# Autodesk Inventor assembly: pld-octogon
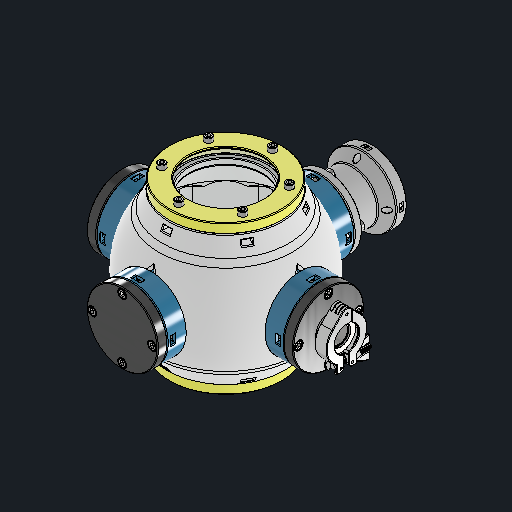
[picture p0: Inventor's stored thumbnail of the model, 512x512]
Saved by Autodesk Inventor 2026 (Build 300175050, 175E)
## iProperties
Created: 2025-12-11
Part Number: pld-octogon
Document SubType Name: Assembly
Designer: kuzmin
Author: kuzmin
## Documents named in this file (11)
- C:\Users\queezz\Dropbox\Drawings\PIHTI\PLD\pld-octogon.iam
- C:\Users\queezz\Dropbox\Drawings\PIHTI\PLD\pld-octogon.ipt
- C:\Users\queezz\Dropbox\Drawings\PIHTI\PLD\pld-octogon-nipple.ipt
- C:\Users\queezz\Dropbox\Drawings\PIHTI\PLD\oring-60-68.ipt
- C:\Users\queezz\Dropbox\Drawings\PIHTI\PLD\pld_nipple-70mm.iam
- C:\Users\queezz\Dropbox\Drawings\PIHTI\ContentCenter\Fastners\M6-nut-WA5.ipt
- C:\Users\queezz\Dropbox\Drawings\PIHTI\ContentCenter\Fastners\M6x25-SHCS.ipt
- C:\Users\queezz\Dropbox\Drawings\PIHTI\PLD\oring-102-110.ipt
- C:\Users\queezz\Dropbox\Drawings\PIHTI\PLD\akf-100-window.iam
- C:\Users\queezz\Dropbox\Drawings\PIHTI\PLD\akf-60-blank.ipt
- C:\Users\queezz\Dropbox\Drawings\PIHTI\PLD\akf-60-nw25.iam
## Components (47 placed, 10 different names)
1. pld-octogon:1 — Rigid:1, Flush:1, Flush:2, Mate:1, Rigid:3, Rigid:4, Rigid:5, Rigid:18, Rigid:19, Rigid:26, Rotational:1, Rigid:33, Rigid:34, Rigid:35, Rigid:36, Rigid:37, Rigid:38
2. pld-octogon-nipple:1 — Rigid:1, Rigid:6, Mate:2, Mate:3
3. pld-octogon-nipple:2 — Rigid:3
4. pld-octogon-nipple:3 — Rigid:4
5. pld-octogon-nipple:4 — Rigid:5
6. oring-60-68:1 — Rigid:6, Tangent:1
7. oring-60-68:2
8. oring-60-68:3
9. oring-60-68:4
10. pld_nipple-70mm:1 [sub-assembly] — Mate:2, Mate:3, Tangent:1, Rigid:14, Rigid:15, Rigid:16, Rigid:17
11. oring-102-110:1 — Rigid:18
12. akf-100-window:2 [sub-assembly] — Rigid:19, Rigid:20, Rigid:21, Rigid:22, Rigid:23, Rigid:24, Rigid:25
13. akf-100-window:3 [sub-assembly] — Rotational:1, Rigid:27, Rigid:28, Rigid:29, Rigid:30, Rigid:31, Rigid:32
14. oring-102-110:2 — Rigid:26
15. akf-60-blank:2 — Rigid:44, Rigid:45, Rigid:46, Rigid:47
16. akf-60-blank:3
17. akf-60-nw25:2 [sub-assembly]
18. IS 2269 M6 x 25:17 — Rigid:47
19. IS 2269 M6 x 25:18 — Rigid:44
20. IS 2269 M6 x 25:19 — Rigid:46
21. IS 2269 M6 x 25:20 — Rigid:45
22. JIS B 1181 -finished Class 1 - Metric Class 1 -finishedM6:5 — Rigid:33
23. JIS B 1181 -finished Class 1 - Metric Class 1 -finishedM6:6 — Rigid:38
24. JIS B 1181 -finished Class 1 - Metric Class 1 -finishedM6:7 — Rigid:36
25. JIS B 1181 -finished Class 1 - Metric Class 1 -finishedM6:8 — Rigid:34
26. JIS B 1181 -finished Class 1 - Metric Class 1 -finishedM6:9 — Rigid:37
27. JIS B 1181 -finished Class 1 - Metric Class 1 -finishedM6:10 — Rigid:35
28. IS 2269 M6 x 25:11 — Rigid:27
29. IS 2269 M6 x 25:12 — Rigid:31
30. IS 2269 M6 x 25:13 — Rigid:32
31. IS 2269 M6 x 25:14 — Rigid:30
32. IS 2269 M6 x 25:15 — Rigid:29
33. IS 2269 M6 x 25:16 — Rigid:28
34. IS 2269 M6 x 25:5 — Rigid:21
35. IS 2269 M6 x 25:6 — Rigid:22
36. IS 2269 M6 x 25:7 — Rigid:23
37. IS 2269 M6 x 25:8 — Rigid:25
38. IS 2269 M6 x 25:9 — Rigid:24
39. IS 2269 M6 x 25:10 — Rigid:20
40. JIS B 1181 -finished Class 1 - Metric Class 1 -finishedM6:1
41. JIS B 1181 -finished Class 1 - Metric Class 1 -finishedM6:2
42. JIS B 1181 -finished Class 1 - Metric Class 1 -finishedM6:3
43. JIS B 1181 -finished Class 1 - Metric Class 1 -finishedM6:4
44. IS 2269 M6 x 25:1 — Rigid:16
45. IS 2269 M6 x 25:2 — Rigid:17
46. IS 2269 M6 x 25:3 — Rigid:15
47. IS 2269 M6 x 25:4 — Rigid:14
## Relationships (42: WeldJoint 35, Mate 3, Flush 2, Tangent 1, RevoluteJoint 1)
- Rigid:1 [WeldJoint] (2.8 mm): pld-octogon:1 ↔ pld-octogon-nipple:1
- Flush:1: pld-octogon:1
- Flush:2: pld-octogon:1
- Mate:1: pld-octogon:1
- Rigid:3 [WeldJoint] (-3 mm): pld-octogon:1 ↔ pld-octogon-nipple:2
- Rigid:4 [WeldJoint] (-3 mm): pld-octogon:1 ↔ pld-octogon-nipple:3
- Rigid:5 [WeldJoint] (1 mm): pld-octogon:1 ↔ pld-octogon-nipple:4
- Rigid:6 [WeldJoint] (2 mm): pld-octogon-nipple:1 ↔ oring-60-68:1
- Mate:2: pld-octogon-nipple:1 ↔ pld_nipple-70mm:1
- Mate:3: pld-octogon-nipple:1 ↔ pld_nipple-70mm:1
- Tangent:1: oring-60-68:1 ↔ pld_nipple-70mm:1
- Rigid:14 [WeldJoint]: pld_nipple-70mm:1 ↔ IS 2269 M6 x 25:4
- Rigid:15 [WeldJoint]: pld_nipple-70mm:1 ↔ IS 2269 M6 x 25:3
- Rigid:16 [WeldJoint]: pld_nipple-70mm:1 ↔ IS 2269 M6 x 25:1
- Rigid:17 [WeldJoint]: pld_nipple-70mm:1 ↔ IS 2269 M6 x 25:2
- Rigid:18 [WeldJoint] (2 mm): pld-octogon:1 ↔ oring-102-110:1
- Rigid:19 [WeldJoint]: pld-octogon:1 ↔ akf-100-window:2
- Rigid:20 [WeldJoint]: akf-100-window:2 ↔ IS 2269 M6 x 25:10
- Rigid:21 [WeldJoint]: akf-100-window:2 ↔ IS 2269 M6 x 25:5
- Rigid:22 [WeldJoint]: akf-100-window:2 ↔ IS 2269 M6 x 25:6
- Rigid:23 [WeldJoint]: akf-100-window:2 ↔ IS 2269 M6 x 25:7
- Rigid:24 [WeldJoint]: akf-100-window:2 ↔ IS 2269 M6 x 25:9
- Rigid:25 [WeldJoint]: akf-100-window:2 ↔ IS 2269 M6 x 25:8
- Rigid:26 [WeldJoint] (2 mm): pld-octogon:1 ↔ oring-102-110:2
- Rotational:1 [RevoluteJoint]: pld-octogon:1 ↔ akf-100-window:3
- Rigid:27 [WeldJoint]: akf-100-window:3 ↔ IS 2269 M6 x 25:11
- Rigid:28 [WeldJoint]: akf-100-window:3 ↔ IS 2269 M6 x 25:16
- Rigid:29 [WeldJoint]: akf-100-window:3 ↔ IS 2269 M6 x 25:15
- Rigid:30 [WeldJoint]: akf-100-window:3 ↔ IS 2269 M6 x 25:14
- Rigid:31 [WeldJoint]: akf-100-window:3 ↔ IS 2269 M6 x 25:12
- Rigid:32 [WeldJoint]: akf-100-window:3 ↔ IS 2269 M6 x 25:13
- Rigid:33 [WeldJoint]: pld-octogon:1 ↔ JIS B 1181 -finished Class 1 - Metric Class 1 -finishedM6:5
- Rigid:34 [WeldJoint] (0.6 mm): pld-octogon:1 ↔ JIS B 1181 -finished Class 1 - Metric Class 1 -finishedM6:8
- Rigid:35 [WeldJoint] (0.6 mm): pld-octogon:1 ↔ JIS B 1181 -finished Class 1 - Metric Class 1 -finishedM6:10
- Rigid:36 [WeldJoint]: pld-octogon:1 ↔ JIS B 1181 -finished Class 1 - Metric Class 1 -finishedM6:7
- Rigid:37 [WeldJoint] (0.6 mm): pld-octogon:1 ↔ JIS B 1181 -finished Class 1 - Metric Class 1 -finishedM6:9
- Rigid:38 [WeldJoint]: pld-octogon:1 ↔ JIS B 1181 -finished Class 1 - Metric Class 1 -finishedM6:6
- [WeldJoint]: pld-octogon-nipple:2 ↔ akf-60-nw25:2
- Rigid:44 [WeldJoint]: akf-60-blank:2 ↔ IS 2269 M6 x 25:18
- Rigid:45 [WeldJoint] (0.3 mm): akf-60-blank:2 ↔ IS 2269 M6 x 25:20
- Rigid:46 [WeldJoint] (0.3 mm): akf-60-blank:2 ↔ IS 2269 M6 x 25:19
- Rigid:47 [WeldJoint] (0.3 mm): akf-60-blank:2 ↔ IS 2269 M6 x 25:17
